# Autodesk Inventor assembly: Puller Mechnaism
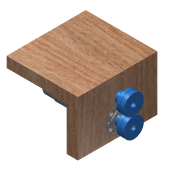
[picture p0: Inventor's stored thumbnail of the model, 180x180]
Saved by Autodesk Inventor 2014 SP1 (Build 180222100, 222)
## iProperties
Created: 2014-11-18
Part Number: Puller Mechnaism
Document SubType Name: Assembly
Designer: AlecShufelt
Author: AlecShufelt
## Documents named in this file (5)
- C:\Users\AlecShufelt\Documents\Drafting\CEMS Research\Prototype 2.0\Puller Mechnaism.iam
- C:\Users\AlecShufelt\Documents\Drafting\CEMS Research\Prototype 2.0\Puller Wheel.ipt
- C:\Users\AlecShufelt\Documents\Drafting\CEMS Research\Prototype 2.0\Rubber Band.ipt
- C:\Users\AlecShufelt\Documents\Drafting\CEMS Research\Prototype 2.0\Pulling Bracket.ipt
- C:\Users\AlecShufelt\Documents\Drafting\CEMS Research\Prototype 2.0\Imported Components\PG-71-am-0914\PG-71-am-0914.ipt
## Components (5 placed, 4 different names)
1. Puller Wheel:1 — Flush:1, Flush:2, Tangent:1, Tangent:2, Mate:1
2. Puller Wheel:2 — Flush:1, Flush:2, Tangent:1, Tangent:3
3. PG-71-am-0914:3
4. Rubber Band:1 — Tangent:2, Mate:1, Tangent:3
5. Pulling Bracket:1
## Relationships (8: Tangent 3, Flush 2, Insert 2, Mate 1)
- Flush:1: Puller Wheel:1 ↔ Puller Wheel:2
- Flush:2: Puller Wheel:1 ↔ Puller Wheel:2
- [Insert] (-22.86 mm): Puller Wheel:2 ↔ PG-71-am-0914:3
- Tangent:1: Puller Wheel:1 ↔ Puller Wheel:2
- Tangent:2: Puller Wheel:1 ↔ Rubber Band:1
- Mate:1: Puller Wheel:1 ↔ Rubber Band:1
- Tangent:3: Puller Wheel:2 ↔ Rubber Band:1
- [Insert]: PG-71-am-0914:3 ↔ Pulling Bracket:1
